# Autodesk Inventor assembly: Tenor Cart OPTION 2
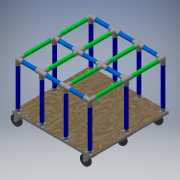
[picture p0: Inventor's stored thumbnail of the model, 180x180]
Saved by Autodesk Inventor 2018.2 (Build 222227000, 227)
## iProperties
Created: 2018-03-15
Part Number: Tenor Cart OPTION 2
Document SubType Name: Assembly
Designer: owner
Author: owner
## Documents named in this file (10)
- Z:\The Pickle - 4 - Copy\Final Carts\Sax Cart\Tenor Sax Cart.iam
- Z:\The Pickle - 4 - Copy\Final Carts\Sax Cart\Tenor Plywood Base.ipt
- Z:\The Pickle - 4 - Copy\Final Carts\Sax Cart\Sax Pipe 1 (Tenor and Bari).ipt
- Z:\The Pickle - 4 - Copy\Final Carts\Sax Cart\Sax Pipe 2 (Tenor and Bari).ipt
- Z:\The Pickle - 4 - Copy\Final Carts\Stuff Used By All Carts\PVC Fittings (Formufit)\Wood Mount 1 Inch.ipt
- Z:\The Pickle - 4 - Copy\Final Carts\Stuff Used By All Carts\PVC Fittings (Formufit)\3-way 90 1 Inch.ipt
- Z:\The Pickle - 4 - Copy\Final Carts\Stuff Used By All Carts\PVC Fittings (Formufit)\4-way Tee 1 Inch.ipt
- Z:\The Pickle - 4 - Copy\Final Carts\Stuff Used By All Carts\PVC Fittings (Formufit)\Cross 1 Inch.ipt
- Z:\The Pickle - 4 - Copy\Final Carts\Stuff Used By All Carts\WHEELS.ipt
- Z:\The Pickle - 4 - Copy\Final Carts\Sax Cart\Tenor Sax Pipe 3.ipt
## Components (56 placed, 9 different names)
1. Tenor Plywood Base:1 — Mate:1, Tangent:1, Tangent:2, Tangent:3, Flush:28, Flush:29, Mate:2, Flush:30, Flush:31, Tangent:4, Tangent:5, Tangent:6, Tangent:7, Angle:1
2. Tenor Sax Pipe 3:1 — Insert:10, Insert:73, Tangent:8
3. Tenor Sax Pipe 3:2 — Insert:69, Insert:72
4. Tenor Sax Pipe 3:3 — Insert:23
5. Tenor Sax Pipe 3:4 — Insert:24, Insert:29
6. Sax Pipe 1 (Tenor and Bari):1 — Insert:1, Insert:9
7. Sax Pipe 1 (Tenor and Bari):2 — Insert:2, Insert:68
8. Sax Pipe 1 (Tenor and Bari):5 — Insert:5, Insert:64
9. Sax Pipe 2 (Tenor and Bari):1 — Insert:30
10. Sax Pipe 2 (Tenor and Bari):2 — Insert:74
11. Sax Pipe 2 (Tenor and Bari):3 — Insert:71
12. Sax Pipe 2 (Tenor and Bari):4
13. Sax Pipe 2 (Tenor and Bari):5 — Insert:37
14. Sax Pipe 2 (Tenor and Bari):6 — Insert:31
15. Sax Pipe 1 (Tenor and Bari):8 — Insert:4, Insert:25, Mate:3
16. Wood Mount 1 Inch:1 — Flush:7, Mate:1, Tangent:1, Tangent:2, Tangent:3, Insert:1
17. Wood Mount 1 Inch:2 — Flush:6, Flush:7, Insert:4
18. Wood Mount 1 Inch:3 — Flush:6, Insert:5, Tangent:4
19. Wood Mount 1 Inch:8 — Insert:2, Tangent:6
20. 3-way 90 1 Inch:1 — Insert:47, Insert:48, Insert:50
21. 3-way 90 1 Inch:2 — Insert:56, Insert:57, Insert:58
22. 3-way 90 1 Inch:3 — Insert:63, Insert:64
23. 3-way 90 1 Inch:4 — Insert:9, Insert:10, Insert:30
24. 4-way Tee 1 Inch:1 — Insert:25, Insert:29, Insert:31
25. 4-way Tee 1 Inch:3 — Insert:51, Insert:52, Insert:53, Insert:55
26. Cross 1 Inch:2 — Insert:23, Insert:24, Insert:37
27. WHEELS:1 — Flush:8, Flush:15, Flush:21, Flush:29, Mate:2
28. WHEELS:2 — Flush:9, Flush:15, Flush:16, Flush:22, Mate:3
29. WHEELS:3 — Flush:10, Flush:16, Flush:23
30. WHEELS:6 — Flush:10, Flush:13, Flush:19, Flush:23, Flush:30, Flush:31
31. WHEELS:7 — Flush:9, Flush:12, Flush:13, Flush:18, Flush:19, Flush:22
32. WHEELS:8 — Flush:8, Flush:12, Flush:18, Flush:21, Flush:28
33. Tenor Sax Pipe 3:5 — Insert:47, Insert:70
34. Tenor Sax Pipe 3:6 — Insert:53, Insert:54
35. Tenor Sax Pipe 3:7 — Insert:57, Insert:78
36. Tenor Sax Pipe 3:8 — Insert:76, Insert:77
37. Tenor Sax Pipe 3:9 — Insert:63, Insert:75
38. Sax Pipe 2 (Tenor and Bari):7 — Insert:50, Insert:51
39. Sax Pipe 2 (Tenor and Bari):8 — Insert:55, Insert:56
40. Sax Pipe 1 (Tenor and Bari):9 — Insert:48
41. Wood Mount 1 Inch:9
42. Sax Pipe 1 (Tenor and Bari):10 — Insert:52
43. Wood Mount 1 Inch:10
44. Sax Pipe 1 (Tenor and Bari):11 — Insert:58
45. Wood Mount 1 Inch:11 — Tangent:7
46. Sax Pipe 1 (Tenor and Bari):12 — Insert:67
47. Wood Mount 1 Inch:12 — Tangent:5
48. Sax Pipe 1 (Tenor and Bari):13 — Insert:66
49. Wood Mount 1 Inch:13
50. Sax Pipe 1 (Tenor and Bari):14 — Insert:65
51. Wood Mount 1 Inch:14
52. Cross 1 Inch:3 — Insert:54
53. 4-way Tee 1 Inch:4 — Insert:65, Insert:69, Insert:70, Insert:71
54. 4-way Tee 1 Inch:5 — Insert:66, Insert:72, Insert:73, Insert:74
55. 4-way Tee 1 Inch:6 — Insert:67, Insert:75, Insert:76
56. 4-way Tee 1 Inch:7 — Insert:68, Insert:77, Insert:78
## Relationships (76: Insert 46, Flush 18, Tangent 8, Mate 3, Angle 1)
- Flush:6: Wood Mount 1 Inch:2 ↔ Wood Mount 1 Inch:3
- Flush:7: Wood Mount 1 Inch:1 ↔ Wood Mount 1 Inch:2
- Mate:1: Tenor Plywood Base:1 ↔ Wood Mount 1 Inch:1
- Tangent:1: Tenor Plywood Base:1 ↔ Wood Mount 1 Inch:1
- Tangent:2: Tenor Plywood Base:1 ↔ Wood Mount 1 Inch:1
- Tangent:3: Tenor Plywood Base:1 ↔ Wood Mount 1 Inch:1
- Insert:1: Sax Pipe 1 (Tenor and Bari):1 ↔ Wood Mount 1 Inch:1
- Insert:2: Sax Pipe 1 (Tenor and Bari):2 ↔ Wood Mount 1 Inch:8
- Insert:4: Sax Pipe 1 (Tenor and Bari):8 ↔ Wood Mount 1 Inch:2
- Insert:5: Sax Pipe 1 (Tenor and Bari):5 ↔ Wood Mount 1 Inch:3
- Insert:9: Sax Pipe 1 (Tenor and Bari):1 ↔ 3-way 90 1 Inch:4
- Insert:10: Tenor Sax Pipe 3:1 ↔ 3-way 90 1 Inch:4
- Insert:23: Tenor Sax Pipe 3:3 ↔ Cross 1 Inch:2
- Insert:24: Tenor Sax Pipe 3:4 ↔ Cross 1 Inch:2
- Insert:25: Sax Pipe 1 (Tenor and Bari):8 ↔ 4-way Tee 1 Inch:1
- Insert:29: Tenor Sax Pipe 3:4 ↔ 4-way Tee 1 Inch:1
- Insert:30: Sax Pipe 2 (Tenor and Bari):1 ↔ 3-way 90 1 Inch:4
- Insert:31: Sax Pipe 2 (Tenor and Bari):6 ↔ 4-way Tee 1 Inch:1
- Insert:37: Sax Pipe 2 (Tenor and Bari):5 ↔ Cross 1 Inch:2
- Flush:8: WHEELS:1 ↔ WHEELS:8
- Flush:9: WHEELS:2 ↔ WHEELS:7
- Flush:10: WHEELS:3 ↔ WHEELS:6
- Flush:12: WHEELS:7 ↔ WHEELS:8
- Flush:13: WHEELS:6 ↔ WHEELS:7
- Flush:15: WHEELS:1 ↔ WHEELS:2
- Flush:16: WHEELS:2 ↔ WHEELS:3
- Flush:18: WHEELS:7 ↔ WHEELS:8
- Flush:19: WHEELS:6 ↔ WHEELS:7
- Flush:21: WHEELS:1 ↔ WHEELS:8
- Flush:22: WHEELS:2 ↔ WHEELS:7
- Flush:23: WHEELS:3 ↔ WHEELS:6
- Flush:28: Tenor Plywood Base:1 ↔ WHEELS:8
- Flush:29: Tenor Plywood Base:1 ↔ WHEELS:1
- Mate:2: Tenor Plywood Base:1 ↔ WHEELS:1
- [Insert]: Sax Pipe 1 (Tenor and Bari):9 ↔ Wood Mount 1 Inch:9
- [Insert]: Sax Pipe 1 (Tenor and Bari):10 ↔ Wood Mount 1 Inch:10
- [Insert]: Sax Pipe 1 (Tenor and Bari):11 ↔ Wood Mount 1 Inch:11
- [Insert]: Sax Pipe 1 (Tenor and Bari):12 ↔ Wood Mount 1 Inch:12
- [Insert]: Sax Pipe 1 (Tenor and Bari):13 ↔ Wood Mount 1 Inch:13
- [Insert]: Sax Pipe 1 (Tenor and Bari):14 ↔ Wood Mount 1 Inch:14
- Insert:47: 3-way 90 1 Inch:1 ↔ Tenor Sax Pipe 3:5
- Insert:48: 3-way 90 1 Inch:1 ↔ Sax Pipe 1 (Tenor and Bari):9
- Insert:50: 3-way 90 1 Inch:1 ↔ Sax Pipe 2 (Tenor and Bari):7
- Insert:51: 4-way Tee 1 Inch:3 ↔ Sax Pipe 2 (Tenor and Bari):7
- Insert:52: 4-way Tee 1 Inch:3 ↔ Sax Pipe 1 (Tenor and Bari):10
- Insert:53: 4-way Tee 1 Inch:3 ↔ Tenor Sax Pipe 3:6
- Insert:54: Tenor Sax Pipe 3:6 ↔ Cross 1 Inch:3
- Insert:55: 4-way Tee 1 Inch:3 ↔ Sax Pipe 2 (Tenor and Bari):8
- Insert:56: 3-way 90 1 Inch:2 ↔ Sax Pipe 2 (Tenor and Bari):8
- Insert:57: 3-way 90 1 Inch:2 ↔ Tenor Sax Pipe 3:7
- Insert:58: 3-way 90 1 Inch:2 ↔ Sax Pipe 1 (Tenor and Bari):11
- Insert:63: 3-way 90 1 Inch:3 ↔ Tenor Sax Pipe 3:9
- Insert:64: Sax Pipe 1 (Tenor and Bari):5 ↔ 3-way 90 1 Inch:3
- Insert:65: Sax Pipe 1 (Tenor and Bari):14 ↔ 4-way Tee 1 Inch:4
- Insert:66: Sax Pipe 1 (Tenor and Bari):13 ↔ 4-way Tee 1 Inch:5
- Insert:67: Sax Pipe 1 (Tenor and Bari):12 ↔ 4-way Tee 1 Inch:6
- Insert:68: Sax Pipe 1 (Tenor and Bari):2 ↔ 4-way Tee 1 Inch:7
- Insert:69: Tenor Sax Pipe 3:2 ↔ 4-way Tee 1 Inch:4
- Insert:70: Tenor Sax Pipe 3:5 ↔ 4-way Tee 1 Inch:4
- Insert:71: Sax Pipe 2 (Tenor and Bari):3 ↔ 4-way Tee 1 Inch:4
- Insert:72: Tenor Sax Pipe 3:2 ↔ 4-way Tee 1 Inch:5
- Insert:73: Tenor Sax Pipe 3:1 ↔ 4-way Tee 1 Inch:5
- Insert:74: Sax Pipe 2 (Tenor and Bari):2 ↔ 4-way Tee 1 Inch:5
- Insert:75: Tenor Sax Pipe 3:9 ↔ 4-way Tee 1 Inch:6
- Insert:76: Tenor Sax Pipe 3:8 ↔ 4-way Tee 1 Inch:6
- Insert:77: Tenor Sax Pipe 3:8 ↔ 4-way Tee 1 Inch:7
- Insert:78: Tenor Sax Pipe 3:7 ↔ 4-way Tee 1 Inch:7
- Flush:30: Tenor Plywood Base:1 ↔ WHEELS:6
- Flush:31: Tenor Plywood Base:1 ↔ WHEELS:6
- Tangent:4: Tenor Plywood Base:1 ↔ Wood Mount 1 Inch:3
- Tangent:5: Tenor Plywood Base:1 ↔ Wood Mount 1 Inch:12
- Tangent:6: Tenor Plywood Base:1 ↔ Wood Mount 1 Inch:8
- Tangent:7: Tenor Plywood Base:1 ↔ Wood Mount 1 Inch:11
- Mate:3 (-31.75 mm): Sax Pipe 1 (Tenor and Bari):8 ↔ WHEELS:2
- Angle:1 (0 deg): Tenor Plywood Base:1
- Tangent:8: Tenor Sax Pipe 3:1
## Named parameters: d79_d11 = 0 mm, d80_d11 = 0 mm, d81_d11 = 0 mm, d82_d11 = 0 mm, d83_d11 = 0 mm, d84_d11 = 0 mm
